# Autodesk Inventor assembly: LegStart_MIR
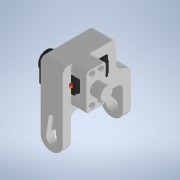
[picture p0: Inventor's stored thumbnail of the model, 180x180]
Saved by Autodesk Inventor 2020.3 (Build 243373000, 373)
## iProperties
Created: 2022-03-31
Part Number: LegStart_MIR
Document SubType Name: Assembly
Designer: sanyi
Author: sanyi
## Documents named in this file (4)
- C:\Users\sanyi\Documents\Inventor\Quadropod\Quadropod MDL\SimulationModell_Assembly\LegStart_MIR.iam
- C:\Users\sanyi\Documents\Inventor\Quadropod\LegPin_v1.ipt
- C:\Users\sanyi\Documents\Inventor\Quadropod\LegStart_v1_MIR1.ipt
- C:\Users\sanyi\Documents\Inventor\Quadropod\SH-0257MG.ipt
## Components (3 placed, 3 different names)
1. LegPin_v1:1 — Insert:1, Insert:2, Mate:4
2. LegStart_v1_MIR1:1 — Insert:1, Insert:2, Insert:3, Angle:1, Angle:2, Mate:5, Mate:6
3. SH-0257MG:1 — Insert:3, Angle:1
## Relationships (9: Insert 3, Mate 3, Angle 2, Flush 1)
- Insert:1: LegPin_v1:1 ↔ LegStart_v1_MIR1:1
- Insert:2: LegPin_v1:1 ↔ LegStart_v1_MIR1:1
- Insert:3: LegStart_v1_MIR1:1 ↔ SH-0257MG:1
- Angle:1 (0 deg): LegStart_v1_MIR1:1 ↔ SH-0257MG:1
- Mate:4: LegPin_v1:1
- Angle:2 (90 deg): LegStart_v1_MIR1:1
- Flush:1
- Mate:5: LegStart_v1_MIR1:1
- Mate:6: LegStart_v1_MIR1:1
